# Autodesk Inventor assembly: PanelJigAssembly_Front
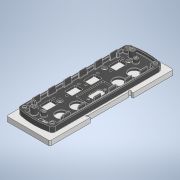
[picture p0: Inventor's stored thumbnail of the model, 180x180]
Saved by Autodesk Inventor 2021 (Build 250183000, 183)
## iProperties
Created: 2020-07-26
Part Number: PanelJigAssembly_Front
Document SubType Name: Assembly
Designer: CASE-SMALL2
Author: CASE-SMALL2
## Documents named in this file (3)
- C:\Users\CASE-SMALL2\Google Drive\Unicorn 2020\CAD_V2\Manufacturing\PanelJigAssembly_Front.iam
- C:\Users\CASE-SMALL2\Google Drive\Unicorn 2020\CAD_V2\Manufacturing\PanelJig.ipt
- C:\Users\CASE-SMALL2\Google Drive\Unicorn 2020\CAD_V2\Front_Panel\Panel\1009799_3D_Front.ipt
## Components (2 placed, 2 different names)
1. PanelJig:1 — Rigid:1
2. 1009799_3D_Front:1 — Rigid:1
## Relationships (1: WeldJoint 1)
- Rigid:1 [WeldJoint]: PanelJig:1 ↔ 1009799_3D_Front:1
